# Autodesk Inventor assembly: halfdrivetrain
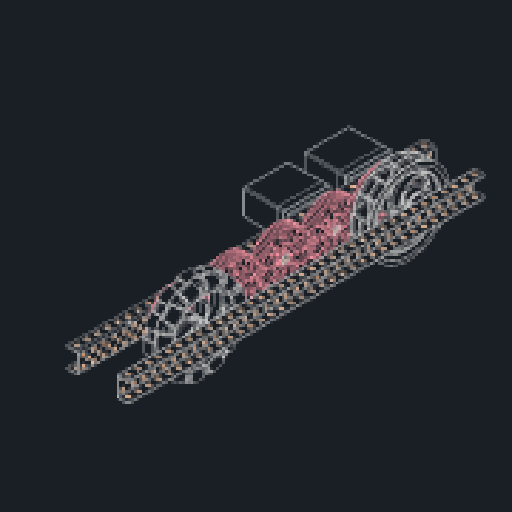
[picture p0: Inventor's stored thumbnail of the model, 512x512]
Saved by Autodesk Inventor 2023 (Build 270158000, 158)
## iProperties
Created: 2023-03-08
Part Number: halfdrivetrain
Document SubType Name: Assembly
Designer: Windows Macbook
Author: Windows Macbook
## Documents named in this file (9)
- C:\Users\Windows Macbook\Desktop\VRC-SPIN-UP\Inventor\Assembly\Pre Worlds\V1\halfdrivetrain.iam
- C:\Users\Windows Macbook\Desktop\VRC-SPIN-UP\Inventor\Structure\C Channel\Aluminum 1x2x1\Alu C 1x2x1x35.ipt
- C:\Users\Windows Macbook\Desktop\VRC-SPIN-UP\Inventor\Assembly\Pre Worlds\V1\omni.iam
- C:\Users\Windows Macbook\Desktop\VRC-SPIN-UP\Inventor\Assembly\Pre Worlds\V1\traction.iam
- C:\Users\Windows Macbook\Desktop\VRC-SPIN-UP\Inventor\Motion\Gears\HS Gear.iam
- C:\Users\Windows Macbook\Desktop\VRC-SPIN-UP\Inventor\Motion\Spacers\Spacer Nylon .313 OD\NSpacer .313 OD x .125.ipt
- C:\Users\Windows Macbook\Desktop\VRC-SPIN-UP\Inventor\Motion\Spacers\Spacer Nylon .313 OD.ipt
- C:\Users\Windows Macbook\Desktop\VRC-SPIN-UP\Inventor\Electronics\V5 Simple Motor.ipt
- C:\Users\Windows Macbook\Desktop\VRC-SPIN-UP\Inventor\Motion\Gears\HS Gear\HS 60T Gear, Square.iam
## Components (13 placed, 6 different names)
1. Alu C 1x2x1x35:1
2. Alu C 1x2x1x35:2 — Insert:2, Insert:24, Insert:26, Insert:30, Insert:31, Insert:32
3. omni:1 [sub-assembly] — Insert:2
4. traction:1 [sub-assembly]
5. V5 Simple Motor:1
6. V5 Simple Motor:2
7. HS 60T Gear, Square:5 [sub-assembly] — Insert:25
8. HS 60T Gear, Square:6 [sub-assembly] — Insert:23
9. NSpacer .313 OD x .125:4 — Insert:23, Insert:24
10. NSpacer .313 OD x .125:5 — Insert:25, Insert:26
11. HS 60T Gear, Square:7 [sub-assembly]
12. NSpacer .313 OD x .125:6 — Insert:30
13. V5 Simple Motor:3 — Insert:31, Insert:32
## Relationships (14: Insert 14)
- [Insert]: Alu C 1x2x1x35:2 ↔ traction:1
- Insert:2: Alu C 1x2x1x35:2 ↔ omni:1
- [Insert]: Alu C 1x2x1x35:2 ↔ V5 Simple Motor:1
- [Insert]: Alu C 1x2x1x35:2 ↔ V5 Simple Motor:1
- [Insert]: Alu C 1x2x1x35:2 ↔ V5 Simple Motor:2
- [Insert]: Alu C 1x2x1x35:2 ↔ V5 Simple Motor:2
- Insert:23: HS 60T Gear, Square:6 ↔ NSpacer .313 OD x .125:4
- Insert:24: Alu C 1x2x1x35:2 ↔ NSpacer .313 OD x .125:4
- Insert:25: HS 60T Gear, Square:5 ↔ NSpacer .313 OD x .125:5
- Insert:26: Alu C 1x2x1x35:2 ↔ NSpacer .313 OD x .125:5
- [Insert]: HS 60T Gear, Square:7 ↔ NSpacer .313 OD x .125:6
- Insert:30: Alu C 1x2x1x35:2 ↔ NSpacer .313 OD x .125:6
- Insert:31: Alu C 1x2x1x35:2 ↔ V5 Simple Motor:3
- Insert:32: Alu C 1x2x1x35:2 ↔ V5 Simple Motor:3
## Named parameters: d3_d15 = 0 mm, d4_d16 = 0 mm, d47_d41 = 0 mm
